# Autodesk Inventor assembly: Camera Edit for Cap
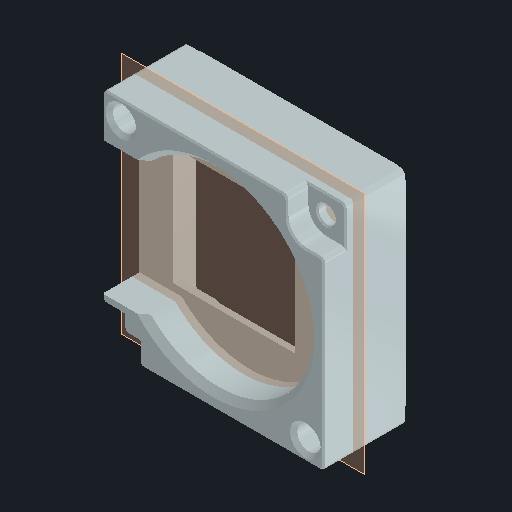
[picture p0: Inventor's stored thumbnail of the model, 512x512]
Saved by Autodesk Inventor 2026 (Build 300175000, 175)
## iProperties
Created: 2023-06-22
Part Number: Camera Edit for Cap
Document SubType Name: Assembly
Designer: FiolkaLab
Sending System: SIEMENS PLM Software NX2206.8900
Preprocessor: ST-DEVELOPER v18.102
Title: STP-MU-(MU196xR-ON+ADPT-MU-CX3-TC-V).stp
## Documents named in this file (2)
- E:\Muaaz\Baseplate\Detection\Camera\Camera Edit for Cap for Machining.iam
- E:\Muaaz\Baseplate\Detection\Camera Edit for Cap\Camera Edit for Cap\MU196-FRONT-KPT.iam
## Components (1 placed, 1 different names)
1. MU196-FRONT-KPT_1017 [sub-assembly] — Flush:1
## Relationships (1: Flush 1)
- Flush:1 (0.8 mm): MU196-FRONT-KPT_1017
